# Autodesk Inventor assembly: battery_status_monitor
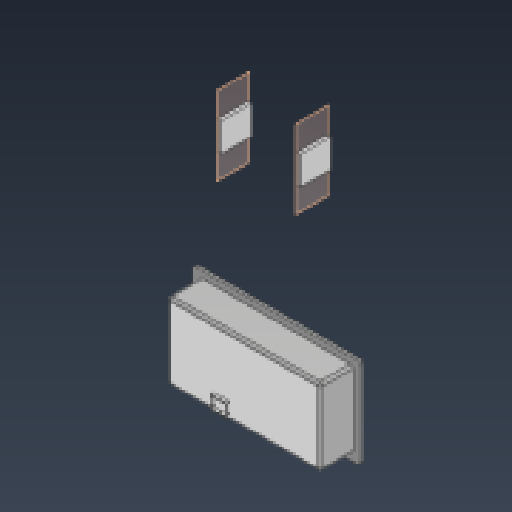
[picture p0: Inventor's stored thumbnail of the model, 512x512]
Saved by Autodesk Inventor 2023 (Build 270158000, 158)
## iProperties
Created: 2025-12-26
Part Number: battery_status_monitor
Document SubType Name: Assembly
Designer: szymo
Author: szymo
## Documents named in this file (3)
- D:\tech\diy\e-skateboard\projekcik-inventor\battery_status_monitor.iam
- D:\tech\diy\e-skateboard\projekcik-inventor\piny_led_bateryjki.ipt
- D:\tech\diy\e-skateboard\projekcik-inventor\DIY.ipt
## Components (3 placed, 2 different names)
1. piny_led_bateryjki:1 — Mate:2, Flush:2, Mate:3
2. piny_led_bateryjki:2 — Mate:1, Flush:1, Mate:4
3. DIY:2 — Mate:1, Mate:2, Flush:1, Flush:2, Mate:3, Mate:4
## Relationships (6: Mate 4, Flush 2)
- Mate:1: piny_led_bateryjki:2 ↔ DIY:2
- Mate:2: piny_led_bateryjki:1 ↔ DIY:2
- Flush:1 (8.75 mm): piny_led_bateryjki:2 ↔ DIY:2
- Flush:2 (-8.75 mm): piny_led_bateryjki:1 ↔ DIY:2
- Mate:3: piny_led_bateryjki:1 ↔ DIY:2
- Mate:4: piny_led_bateryjki:2 ↔ DIY:2
